# Autodesk Inventor assembly: Chasis
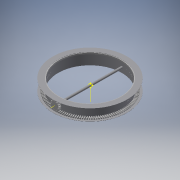
[picture p0: Inventor's stored thumbnail of the model, 180x180]
Saved by Autodesk Inventor 2017 (Build 210142000, 142)
## iProperties
Created: 2016-12-23
Part Number: Chasis
Document SubType Name: Assembly
Designer: David Kopala
Author: David Kopala
## Documents named in this file (5)
- \\Mac\Home\Documents\Drone\Drone\3D Models\Project\Chasis_02\Chasis.iam
- \\Mac\Home\Documents\Drone\Drone\3D Models\Project\Chasis_02\Layer2Assembly.iam
- \\Mac\Home\Documents\Drone\Drone\3D Models\Project\Chasis_02\Bottom_Bevel_Gear.ipt
- \\Mac\Home\Documents\Drone\Drone\3D Models\Project\Chasis_02\Top_Spur_Gear.ipt
- \\Mac\Home\Documents\Drone\Drone\3D Models\Project\Chasis_02\MotorMountAssem.iam
## Components (4 placed, 4 different names)
1. Layer2Assembly:1 [sub-assembly] — Insert:1, Insert:2, Tangent:1, Tangent:2, Tangent:3
2. Bevel Gear1:1 — Insert:1
3. Spur Gear1:1 — Insert:2
4. MotorMountAssem:1 [sub-assembly] — Tangent:1, Tangent:2, Tangent:3
## Relationships (5: Tangent 3, Insert 2)
- Insert:1: Layer2Assembly:1 ↔ Bevel Gear1:1
- Insert:2: Layer2Assembly:1 ↔ Spur Gear1:1
- Tangent:1 (-1.27 mm): Layer2Assembly:1 ↔ MotorMountAssem:1
- Tangent:2 (-1.27 mm): Layer2Assembly:1 ↔ MotorMountAssem:1
- Tangent:3: Layer2Assembly:1 ↔ MotorMountAssem:1
